# Autodesk Inventor assembly: EMU5 Robot
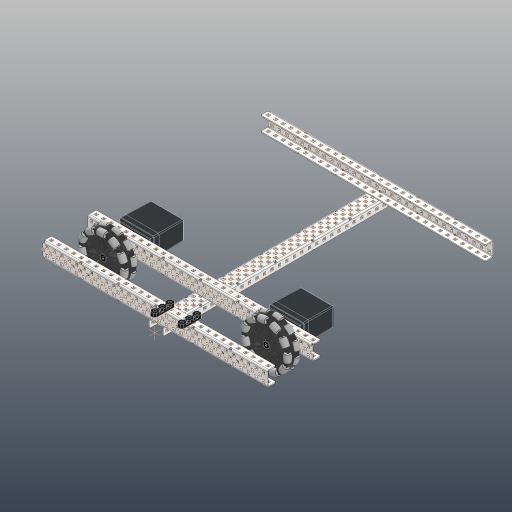
[picture p0: Inventor's stored thumbnail of the model, 512x512]
Saved by Autodesk Inventor 2023 (Build 270158000, 158)
## iProperties
Created: 2022-11-08
Part Number: EMU5 Robot
Document SubType Name: Assembly
Designer: bengo
Author: bengo
## Documents named in this file (6)
- D:\CAD Projects\emu5-15-inch-robot-cad\EMU5 Robot.iam
- D:\VEX CAD Libraries\Inventor\VEX-CAD-Inventor-1.4.0\Structure\C Channel\Aluminum 1x2x1\Alu C 1x2x1x30.ipt
- D:\VEX CAD Libraries\Inventor\VEX-CAD-Inventor-1.4.0\Motion\Shaft LS\Bearing Flat.ipt
- D:\VEX CAD Libraries\Inventor\VEX-CAD-Inventor-1.4.0\Electronics\V5 Simple Motor.ipt
- D:\VEX CAD Libraries\Inventor\VEX-CAD-Inventor-1.4.0\Motion\Wheels\Omni Wheel\3.25 Omni AS, Square.iam
- D:\VEX CAD Libraries\Inventor\VEX-CAD-Inventor-1.4.0\Motion\Wheels\Omni Wheel.iam
## Components (12 placed, 4 different names)
1. Alu C 1x2x1x30:1 — Insert:1, Mate:1, Insert:2, Mate:2, Insert:3, Mate:3
2. Alu C 1x2x1x30:2 — Insert:1, Mate:1, Insert:4, Mate:4, Insert:5, Mate:5
3. Alu C 1x2x1x30:3 — Insert:2, Mate:2
4. Alu C 1x2x1x30:4 — Insert:3, Mate:3, Insert:6, Mate:6, Insert:7, Mate:7
5. Bearing Flat:1
6. Bearing Flat:2 — Insert:4, Mate:4
7. Bearing Flat:3
8. Bearing Flat:4 — Insert:5, Mate:5
9. V5 Simple Motor:1 — Insert:6, Mate:6, Front Left Wheel
10. V5 Simple Motor:2 — Insert:7, Mate:7, Back Left Wheel
11. 3.25 Omni AS, Square:1 [sub-assembly] — Front Left Wheel
12. 3.25 Omni AS, Square:2 [sub-assembly] — Back Left Wheel
## Relationships (16: Insert 9, Mate 7)
- Insert:1: Alu C 1x2x1x30:1 ↔ Alu C 1x2x1x30:2
- Mate:1: Alu C 1x2x1x30:1 ↔ Alu C 1x2x1x30:2
- Insert:2: Alu C 1x2x1x30:1 ↔ Alu C 1x2x1x30:3
- Mate:2: Alu C 1x2x1x30:1 ↔ Alu C 1x2x1x30:3
- Insert:3: Alu C 1x2x1x30:1 ↔ Alu C 1x2x1x30:4
- Mate:3: Alu C 1x2x1x30:1 ↔ Alu C 1x2x1x30:4
- Insert:4: Alu C 1x2x1x30:2 ↔ Bearing Flat:2
- Mate:4: Alu C 1x2x1x30:2 ↔ Bearing Flat:2
- Insert:5: Alu C 1x2x1x30:2 ↔ Bearing Flat:4
- Mate:5: Alu C 1x2x1x30:2 ↔ Bearing Flat:4
- Insert:6: Alu C 1x2x1x30:4 ↔ V5 Simple Motor:1
- Mate:6: Alu C 1x2x1x30:4 ↔ V5 Simple Motor:1
- Insert:7: Alu C 1x2x1x30:4 ↔ V5 Simple Motor:2
- Mate:7: Alu C 1x2x1x30:4 ↔ V5 Simple Motor:2
- Front Left Wheel [Insert] (25.4 mm): V5 Simple Motor:1 ↔ 3.25 Omni AS, Square:1
- Back Left Wheel [Insert] (25.4 mm): V5 Simple Motor:2 ↔ 3.25 Omni AS, Square:2
